# Autodesk Inventor assembly: Pin Support Group
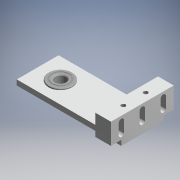
[picture p0: Inventor's stored thumbnail of the model, 180x180]
Saved by Autodesk Inventor 2016 (Build 200138000, 138)
## iProperties
Created: 2015-08-06
Part Number: Pin Support Group
Document SubType Name: Assembly
Designer: Matthew Cheung
Author: Matthew Cheung
## Documents named in this file (4)
- C:\Users\Matthew Cheung\Dropbox\Work\National Instruments\Shared Folder\NI Ball Bearing Slider Crank\CAD\Assemblies\Pin Support Group.iam
- C:\Users\Matthew Cheung\Dropbox\Work\National Instruments\Shared Folder\NI Ball Bearing Slider Crank\CAD\Pin Support Plate.ipt
- C:\Users\Matthew Cheung\Dropbox\Work\National Instruments\Shared Folder\NI Ball Bearing Slider Crank\CAD\Motor Base.ipt
- C:\Users\Matthew Cheung\Dropbox\Work\National Instruments\Shared Folder\NI Ball Bearing Slider Crank\CAD\Bearing - 6384K361.ipt
## Components (3 placed, 3 different names)
1. Pin Support Plate:1 — Mate:3, Mate:4, Mate:5, Mate:6, Mate:7
2. Motor Base:1 — Mate:3, Mate:4, Mate:5
3. Bearing - 6384K361:1 — Mate:6, Mate:7
## Relationships (5: Mate 5)
- Mate:3: Pin Support Plate:1 ↔ Motor Base:1
- Mate:4: Pin Support Plate:1 ↔ Motor Base:1
- Mate:5: Pin Support Plate:1 ↔ Motor Base:1
- Mate:6: Pin Support Plate:1 ↔ Bearing - 6384K361:1
- Mate:7: Pin Support Plate:1 ↔ Bearing - 6384K361:1
